# Autodesk Inventor assembly: akkum
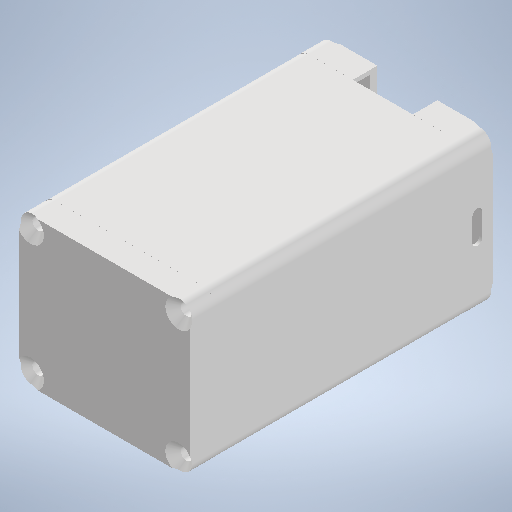
[picture p0: Inventor's stored thumbnail of the model, 512x512]
Saved by Autodesk Inventor 2025 (Build 290162000, 162)
## iProperties
Created: 2026-06-26
Part Number: akkum
Document SubType Name: Assembly
Designer: garin
Author: garin
## Documents named in this file (6)
- C:\Users\garin\Documents\Git\TheseusV2_Maze\Construction\akkum_TSE\akkum.iam
- C:\Users\garin\Documents\Git\TheseusV2_Maze\Construction\akkum_TSE\akkum.ipt
- C:\Users\garin\Documents\Git\TheseusV2_Maze\Construction\akkum_TSE\18650\18650.ipt
- C:\Users\garin\Documents\Git\TheseusV2_Maze\Construction\akkum_TSE\Li-Ion_BMS_4S_20A\Li-Ion_BMS_4S_20A.ipt
- C:\Users\garin\Documents\Git\TheseusV2_Maze\Construction\akkum_TSE\akkum_cap_bms.ipt
- C:\Users\garin\Documents\Git\TheseusV2_Maze\Construction\akkum_TSE\akkum_cap_pd.ipt
## Components (8 placed, 5 different names)
1. akkum:1 — Заподлицо:1, Заподлицо:2, Заподлицо:3, Совмещение:1, Совмещение:2, Совмещение:3, Совмещение:4, Совмещение:5, Совмещение:6, Совмещение:7, Совмещение:8, Совмещение:9, Совмещение:10, Угол:1, Заподлицо:4, Заподлицо:5, Совмещение:11, Совмещение:12, Совмещение:13, Совмещение:14
2. 18650:1 — Совмещение:3, Совмещение:4
3. 18650:2 — Совмещение:7, Совмещение:8
4. 18650:3 — Совмещение:5, Совмещение:6
5. 18650:4 — Совмещение:1, Совмещение:2
6. Li-Ion_BMS_4S_20A:1 — Совмещение:9, Совмещение:10, Угол:1
7. akkum_cap_bms:1 — Заподлицо:4, Совмещение:11, Совмещение:12
8. akkum_cap_pd:1 — Заподлицо:5, Совмещение:13, Совмещение:14
## Relationships (20: Mate 14, Flush 5, Angle 1)
- Заподлицо:1 [Flush]: akkum:1
- Заподлицо:2 [Flush]: akkum:1
- Заподлицо:3 [Flush]: akkum:1
- Совмещение:1 [Mate]: akkum:1 ↔ 18650:4
- Совмещение:2 [Mate]: akkum:1 ↔ 18650:4
- Совмещение:3 [Mate]: akkum:1 ↔ 18650:1
- Совмещение:4 [Mate]: akkum:1 ↔ 18650:1
- Совмещение:5 [Mate]: akkum:1 ↔ 18650:3
- Совмещение:6 [Mate]: akkum:1 ↔ 18650:3
- Совмещение:7 [Mate]: akkum:1 ↔ 18650:2
- Совмещение:8 [Mate]: akkum:1 ↔ 18650:2
- Совмещение:9 [Mate]: akkum:1 ↔ Li-Ion_BMS_4S_20A:1
- Совмещение:10 [Mate]: akkum:1 ↔ Li-Ion_BMS_4S_20A:1
- Угол:1 [Angle] (0 deg): akkum:1 ↔ Li-Ion_BMS_4S_20A:1
- Заподлицо:4 [Flush]: akkum:1 ↔ akkum_cap_bms:1
- Заподлицо:5 [Flush]: akkum:1 ↔ akkum_cap_pd:1
- Совмещение:11 [Mate]: akkum:1 ↔ akkum_cap_bms:1
- Совмещение:12 [Mate]: akkum:1 ↔ akkum_cap_bms:1
- Совмещение:13 [Mate]: akkum:1 ↔ akkum_cap_pd:1
- Совмещение:14 [Mate]: akkum:1 ↔ akkum_cap_pd:1
